# Autodesk Inventor assembly: 3533_20260402144101_8080L+ cover
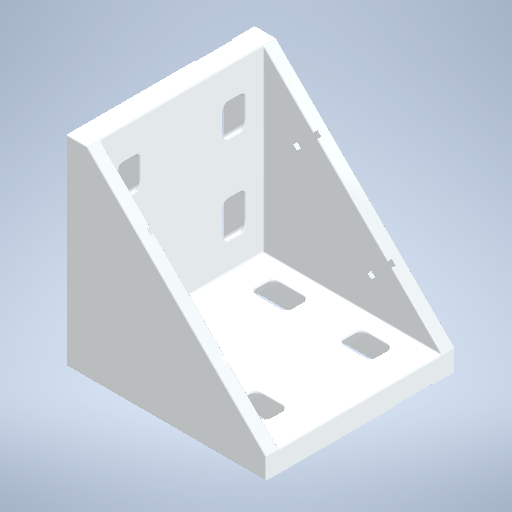
[picture p0: Inventor's stored thumbnail of the model, 512x512]
Saved by Autodesk Inventor 2025.3 (Build 293356000, 356)
## iProperties
Created: 2021-06-03
Part Number: 3533_20260402144101_8080L+ cover
Description: STEP AP214
Document SubType Name: Assembly
Designer: louis
Sending System: SolidWorks 2018
Preprocessor: SwSTEP 2.0
Title: 8080L+ cover.STEP
Revision Number: ANY
## Documents named in this file (3)
- C:\Users\louis\OneDrive\Desktop\R_Trident\02_CAD\01_Standard_Parts\3533_20260402144101_8080L+ cover\A_8080L+ cover.iam
- C:\Users\louis\OneDrive\Desktop\R_Trident\02_CAD\01_Standard_Parts\3533_20260402144101_8080L+ cover\8080L+Cover.ipt
- C:\Users\louis\OneDrive\Desktop\R_Trident\02_CAD\01_Standard_Parts\3533_20260402144101_8080L+ cover\8080L Cover.ipt
## Components (2 placed, 2 different names)
1. 8080L+Cover_1 — Mate:1, Mate:2, Flush:1
2. 8080L Cover_2 — Mate:1, Mate:2, Flush:1
## Relationships (3: Mate 2, Flush 1)
- Mate:1: 8080L+Cover_1 ↔ 8080L Cover_2
- Mate:2: 8080L+Cover_1 ↔ 8080L Cover_2
- Flush:1: 8080L+Cover_1 ↔ 8080L Cover_2
